# Autodesk Inventor assembly: cellSTORM_v5
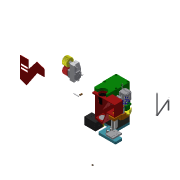
[picture p0: Inventor's stored thumbnail of the model, 180x180]
Saved by Autodesk Inventor 2022 (Build 260153000, 153)
## iProperties
Created: 2020-04-25
Part Number: cellSTORM_v5
Document SubType Name: Assembly
Designer: diederichbenedict
Author: diederichbenedict
## Documents named in this file (20)
- C:\Users\Muriel\Documents\GitHub\cellstorm\INVENTOR\cellSTORM_v6.iam
- C:\Users\Muriel\Documents\GitHub\cellstorm\INVENTOR\00_XY_stage-CHUO_SEIKI_LD-647-R1.iam
- C:\Users\Muriel\Documents\GitHub\cellstorm\INVENTOR\00_Ballmagnets_5mm.ipt
- C:\Users\Muriel\Documents\GitHub\cellstorm\INVENTOR\00_Huawei_P20.ipt
- C:\Users\Muriel\Documents\GitHub\cellstorm\INVENTOR\cellSTORM_Base_v0_R1.ipt
- C:\Users\Muriel\Documents\GitHub\cellstorm\INVENTOR\00_KES400.iam
- C:\Users\Muriel\Documents\GitHub\cellstorm\INVENTOR\cellSTORM_v5_laserstage.ipt
- C:\Users\Muriel\Documents\GitHub\cellstorm\INVENTOR\cellSTORM_v5_cellphonestage.ipt
- C:\Users\Muriel\Documents\GitHub\cellstorm\INVENTOR\cellSTORM_v5_microsocpe.iam
- C:\Users\Muriel\Documents\GitHub\cellstorm\INVENTOR\cellSTORM_v5_microscope_cover.ipt
- C:\Users\Muriel\Documents\GitHub\cellstorm\INVENTOR\00_chip_01_old.ipt
- C:\Users\Muriel\Documents\GitHub\cellstorm\INVENTOR\cellSTORM_v5_chiptray_old_0.ipt
- C:\Users\Muriel\Documents\GitHub\cellstorm\INVENTOR\00_Laser_532nm_200mw.ipt
- C:\Users\Muriel\Documents\GitHub\cellstorm\INVENTOR\00_LN680-Step.ipt
- C:\Users\Muriel\Documents\GitHub\cellstorm\INVENTOR\cellSTORM_v5_motorblock.ipt
- C:\Users\Muriel\Documents\GitHub\cellstorm\INVENTOR\Assembly_Nema_Motor_attachement_for_XYstage.iam
- C:\Users\Muriel\Documents\GitHub\cellstorm\INVENTOR\00_Arduino_CNC_Assembly.iam
- C:\Users\Muriel\Documents\GitHub\cellstorm\INVENTOR\00_LASER_640nm.ipt
- C:\Users\Muriel\Documents\GitHub\cellstorm\INVENTOR\cellSTORM_lightpath.ipt
- C:\Users\diederichbenedict\Dropbox\cellSTORM\cellSTORM_v6.iam
## Components (22 placed, 18 different names)
1. 00_XY_stage-CHUO_SEIKI_LD-647-R1:1 [sub-assembly] — Insert:6, Angle:5, Passend:30, Fluchtend:36, Einfügen:19, Einfügen:20
2. 00_Ballmagnets_5mm:1
3. 00_Ballmagnets_5mm:2
4. 00_Ballmagnets_5mm:3
5. cellSTORM_Base_v0_R1:1 — Fluchtend:36
6. 00_XY_stage-CHUO_SEIKI_LD-647-R1:2 [sub-assembly] — Insert:6, Angle:5, Flush:12, Flush:13, Insert:17
7. cellSTORM_v5_cellphonestage:1 — Flush:12, Flush:13, Flush:29, Fluchtend:33, Fluchtend:34, Fluchtend:35, Fluchtend:37, Passend:36, Winkel:9
8. cellSTORM_v5_microscope_cover:1
9. 00_Huawei_P20:1
10. 00_Laser_532nm_200mw:1
11. 00_LN680-Step:1
12. cellSTORM_v5_motorblock:1 — Flush:29
13. Assembly_Nema_Motor_attachement_for_XYstage:1 [sub-assembly] — Insert:17
14. 00_Arduino_CNC_Assembly:1 [sub-assembly] — Fluchtend:33, Fluchtend:34, Fluchtend:35
15. cellSTORM_v5_laserstage:1 — Einfügen:19, Einfügen:20
16. 00_LASER_640nm:1 — Passend:28, Winkel:8, Passend:32
17. cellSTORM_v5_chiptray_old_0:1 — Passend:33, Passend:34, Passend:35
18. 00_KES400:1 [sub-assembly] — Einfügen:18, Winkel:6, Passend:28, Passend:30, Passend:31, Passend:32, Passend:33, Passend:35
19. 00_chip_01_old:1 — Einfügen:18, Winkel:6, Winkel:8, Passend:34
20. cellSTORM_v5_microsocpe:1 [sub-assembly] — Passend:31, Fluchtend:37, Passend:36, Winkel:9
21. Assembly_Nema_Motor_attachement_for_XYstage:2 [sub-assembly]
22. cellSTORM_lightpath:1
## Relationships (25: Flush 8, Mate 8, Insert 5, Angle 4)
- Insert:6 (6 mm): 00_XY_stage-CHUO_SEIKI_LD-647-R1:1 ↔ 00_XY_stage-CHUO_SEIKI_LD-647-R1:2
- Angle:5 (180 deg): 00_XY_stage-CHUO_SEIKI_LD-647-R1:1 ↔ 00_XY_stage-CHUO_SEIKI_LD-647-R1:2
- Flush:12: 00_XY_stage-CHUO_SEIKI_LD-647-R1:2 ↔ cellSTORM_v5_cellphonestage:1
- Flush:13: 00_XY_stage-CHUO_SEIKI_LD-647-R1:2 ↔ cellSTORM_v5_cellphonestage:1
- Flush:29: cellSTORM_v5_cellphonestage:1 ↔ cellSTORM_v5_motorblock:1
- Insert:17 (10 mm): 00_XY_stage-CHUO_SEIKI_LD-647-R1:2 ↔ Assembly_Nema_Motor_attachement_for_XYstage:1
- Fluchtend:33 [Flush] (12 mm): cellSTORM_v5_cellphonestage:1 ↔ 00_Arduino_CNC_Assembly:1
- Fluchtend:34 [Flush] (-3 mm): cellSTORM_v5_cellphonestage:1 ↔ 00_Arduino_CNC_Assembly:1
- Fluchtend:35 [Flush] (5 mm): cellSTORM_v5_cellphonestage:1 ↔ 00_Arduino_CNC_Assembly:1
- Einfügen:18 [Insert] (1 mm): 00_KES400:1 ↔ 00_chip_01_old:1
- Winkel:6 [Angle] (0 deg): 00_KES400:1 ↔ 00_chip_01_old:1
- Passend:28 [Mate]: 00_LASER_640nm:1 ↔ 00_KES400:1
- Winkel:8 [Angle] (0 deg): 00_LASER_640nm:1 ↔ 00_chip_01_old:1
- Passend:30 [Mate]: 00_XY_stage-CHUO_SEIKI_LD-647-R1:1 ↔ 00_KES400:1
- Passend:31 [Mate]: 00_KES400:1 ↔ cellSTORM_v5_microsocpe:1
- Passend:32 [Mate] (40 mm): 00_LASER_640nm:1 ↔ 00_KES400:1
- Fluchtend:36 [Flush]: 00_XY_stage-CHUO_SEIKI_LD-647-R1:1 ↔ cellSTORM_Base_v0_R1:1
- Passend:33 [Mate]: cellSTORM_v5_chiptray_old_0:1 ↔ 00_KES400:1
- Passend:34 [Mate]: cellSTORM_v5_chiptray_old_0:1 ↔ 00_chip_01_old:1
- Passend:35 [Mate] (3 mm): cellSTORM_v5_chiptray_old_0:1 ↔ 00_KES400:1
- Fluchtend:37 [Flush] (10 mm): cellSTORM_v5_cellphonestage:1 ↔ cellSTORM_v5_microsocpe:1
- Passend:36 [Mate]: cellSTORM_v5_cellphonestage:1 ↔ cellSTORM_v5_microsocpe:1
- Winkel:9 [Angle] (0 deg): cellSTORM_v5_cellphonestage:1 ↔ cellSTORM_v5_microsocpe:1
- Einfügen:19 [Insert]: 00_XY_stage-CHUO_SEIKI_LD-647-R1:1 ↔ cellSTORM_v5_laserstage:1
- Einfügen:20 [Insert]: 00_XY_stage-CHUO_SEIKI_LD-647-R1:1 ↔ cellSTORM_v5_laserstage:1
